# Autodesk Inventor assembly: Oberer Teil
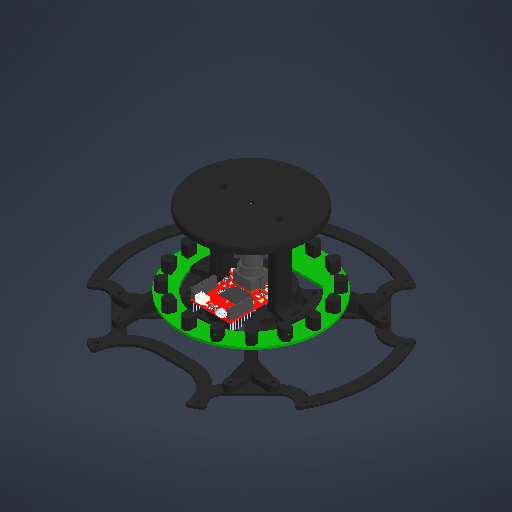
[picture p0: Inventor's stored thumbnail of the model, 512x512]
Saved by Autodesk Inventor 2025.3 (Build 293356000, 356)
## iProperties
Created: 2025-05-27
Part Number: Oberer Teil
Document SubType Name: Assembly
Designer: theod
Author: theod
## Documents named in this file (8)
- C:\Users\theod\Desktop\Robotik Inventor Alles schön\Oberer Teil.iam
- C:\Users\theod\Nextcloud\Inventor\2vs2 LWL Int. 2025\Mittelding mit IR Halterung_1.ipt
- C:\Users\theod\Nextcloud\Inventor\2vs2 LWL Int. 2025\OpenMV Halterung V2.ipt
- C:\Users\theod\Nextcloud\Inventor\2vs2 LWL Int. 2025\openmv-h7-alt\openmv-h7-alt.iam
- C:\Users\theod\Desktop\Robotik Inventor Alles schön\IR_Platine.iam
- C:\Users\theod\Nextcloud\Inventor\2vs2 LWL Int. 2024\Spiegel.ipt
- C:\Users\theod\Downloads\OpenMV Halterung V3.ipt
- C:\Users\theod\Desktop\Team Mathimazierer v2025\Einzelteile\Spiegelhalterung.ipt
## Components (7 placed, 7 different names)
1. Mittelding mit IR Halterung_1:1 — Fluchtend:1, Fluchtend:2, Passend:1, Passend:2, Einfügen:1, Einfügen:2, Passend:10, Passend:11, Passend:12
2. OpenMV Halterung V2:1 — Passend:2, Einfügen:1, Einfügen:2, Einfügen:3, Einfügen:4, Passend:7, Einfügen:5, Einfügen:6
3. openmv-h7-alt:1 [sub-assembly] — Einfügen:3, Einfügen:4
4. IR_Platine:1 [sub-assembly] — Passend:7, Einfügen:5, Einfügen:6
5. Spiegel:1 — Passend:13, Passend:14
6. OpenMV Halterung V3:1 — Passend:10, Passend:11, Passend:12, Einfügen:7, Einfügen:8
7. Spiegelhalterung:1 — Passend:13, Passend:14, Einfügen:7, Einfügen:8
## Relationships (18: Mate 8, Insert 8, Flush 2)
- Fluchtend:1 [Flush]: Mittelding mit IR Halterung_1:1
- Fluchtend:2 [Flush]: Mittelding mit IR Halterung_1:1
- Passend:1 [Mate]: Mittelding mit IR Halterung_1:1
- Passend:2 [Mate]: Mittelding mit IR Halterung_1:1 ↔ OpenMV Halterung V2:1
- Einfügen:1 [Insert]: Mittelding mit IR Halterung_1:1 ↔ OpenMV Halterung V2:1
- Einfügen:2 [Insert]: Mittelding mit IR Halterung_1:1 ↔ OpenMV Halterung V2:1
- Einfügen:3 [Insert]: OpenMV Halterung V2:1 ↔ openmv-h7-alt:1
- Einfügen:4 [Insert]: OpenMV Halterung V2:1 ↔ openmv-h7-alt:1
- Passend:7 [Mate]: OpenMV Halterung V2:1 ↔ IR_Platine:1
- Einfügen:5 [Insert]: OpenMV Halterung V2:1 ↔ IR_Platine:1
- Einfügen:6 [Insert]: OpenMV Halterung V2:1 ↔ IR_Platine:1
- Passend:10 [Mate]: Mittelding mit IR Halterung_1:1 ↔ OpenMV Halterung V3:1
- Passend:11 [Mate]: Mittelding mit IR Halterung_1:1 ↔ OpenMV Halterung V3:1
- Passend:12 [Mate]: Mittelding mit IR Halterung_1:1 ↔ OpenMV Halterung V3:1
- Passend:13 [Mate]: Spiegel:1 ↔ Spiegelhalterung:1
- Passend:14 [Mate]: Spiegel:1 ↔ Spiegelhalterung:1
- Einfügen:7 [Insert]: OpenMV Halterung V3:1 ↔ Spiegelhalterung:1
- Einfügen:8 [Insert]: OpenMV Halterung V3:1 ↔ Spiegelhalterung:1
